# Autodesk Inventor assembly: sensorBoard
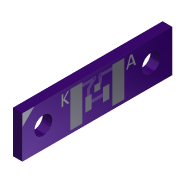
[picture p0: Inventor's stored thumbnail of the model, 180x180]
Saved by Autodesk Inventor 2018.2 (Build 222227000, 227)
## iProperties
Created: 2016-02-15
Part Number: sensorBoard
Document SubType Name: Assembly
Designer: sawai
Author: sawai
## Documents named in this file (3)
- C:\Users\sawaiz\OneDrive\projects\mppcSensor\cad\mppcSensor.iam
- C:\Users\sawaiz\OneDrive\projects\mppcSensor\cad\pcb\pcb.ipt
- C:\Users\sawaiz\OneDrive\projects\mppcSensor\cad\S13360-13xxPE\S13360-13xxPE.iam
## Components (2 placed, 2 different names)
1. pcb:1 — Angle:1, Angle:2, Mate:1
2. S13360-13xxPE:1 [sub-assembly] — Angle:1, Angle:2, Mate:1
## Relationships (3: Angle 2, Mate 1)
- Angle:1 (0 deg): pcb:1 ↔ S13360-13xxPE:1
- Angle:2 (0 deg): pcb:1 ↔ S13360-13xxPE:1
- Mate:1: pcb:1 ↔ S13360-13xxPE:1
